# Autodesk Inventor assembly: MotorMounted
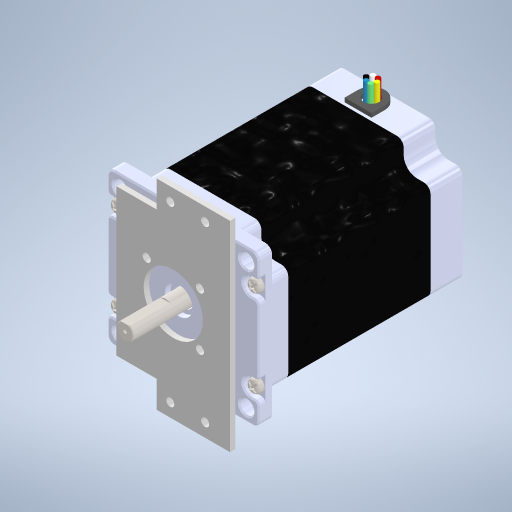
[picture p0: Inventor's stored thumbnail of the model, 512x512]
Saved by Autodesk Inventor 2023 (Build 270158000, 158)
## iProperties
Created: 2024-02-04
Part Number: MotorMounted
Document SubType Name: Assembly
Designer: victo
Author: victo
## Documents named in this file (3)
- C:\Users\victo\Documents\ball-balancing-digital-twin\Mechanics\CAD\MotorMounted.iam
- C:\Users\victo\Documents\ball-balancing-digital-twin\Mechanics\CAD\Step Motor Nema AK23 - 15kg.ipt
- C:\Users\victo\Documents\ball-balancing-digital-twin\Mechanics\CAD\MotorHolder.ipt
## Components (2 placed, 2 different names)
1. Step Motor Nema AK23 - 15kg:1 — Mate:1, Mate:2
2. MotorHolder:1 — Mate:1, Mate:2
## Relationships (2: Mate 2)
- Mate:1: Step Motor Nema AK23 - 15kg:1 ↔ MotorHolder:1
- Mate:2: Step Motor Nema AK23 - 15kg:1 ↔ MotorHolder:1
